# Autodesk Inventor assembly: Servo and Holder
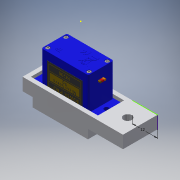
[picture p0: Inventor's stored thumbnail of the model, 180x180]
Saved by Autodesk Inventor 2019 (Build 230136000, 136)
## iProperties
Created: 2022-09-04
Part Number: Servo and Holder
Document SubType Name: Assembly
Designer: Garrett Raker
Author: Garrett Raker
## Documents named in this file (3)
- Z:\ATMAE Robotics\Pill Dispenser Robot\Servo Parts and Assemblies\Servo and Holder.iam
- Z:\ATMAE Robotics\Pill Dispenser Robot\Servo Parts and Assemblies\SG90 360 Degree Servo.ipt
- Z:\ATMAE Robotics\Pill Dispenser Robot\Servo Parts and Assemblies\SG90 360 Degree Servo Holder.ipt
## Components (2 placed, 2 different names)
1. SG90 360 Degree Servo Holder:1 — Mate:1, Mate:2, Mate:3
2. SG90 360 Degree Servo:1 — Mate:1, Mate:2, Mate:3
## Relationships (3: Mate 3)
- Mate:1: SG90 360 Degree Servo Holder:1 ↔ SG90 360 Degree Servo:1
- Mate:2: SG90 360 Degree Servo Holder:1 ↔ SG90 360 Degree Servo:1
- Mate:3: SG90 360 Degree Servo Holder:1 ↔ SG90 360 Degree Servo:1
